# Autodesk Inventor assembly: Motors with Screws
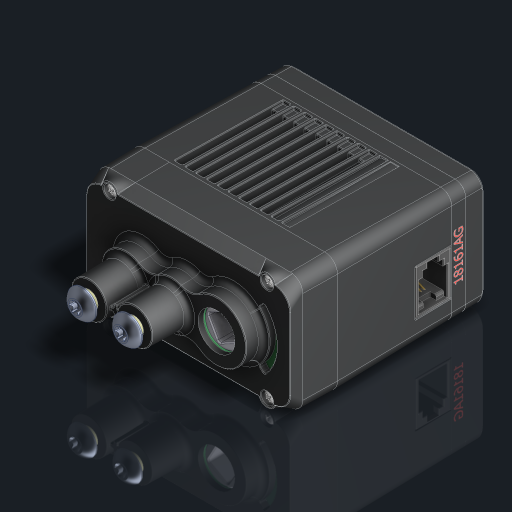
[picture p0: Inventor's stored thumbnail of the model, 512x512]
Saved by Autodesk Inventor 2023.2 (Build 272271030, 271C)
## iProperties
Created: 2022-08-18
Part Number: Motors with Screws
Document SubType Name: Assembly
Designer: ylu12
Author: ylu12
## Documents named in this file (5)
- C:\Users\black\OneDrive\Pictures\Documents\GitHub\New folder\2024-599Z\Cad\Library\VEX-CAD-Inventor-1.4.0\Electronics\Motors with Screws\AluM-StarS.iam
- C:\Users\black\OneDrive\Pictures\Documents\GitHub\New folder\2024-599Z\Cad\Library\VEX-CAD-Inventor-1.4.0\Electronics\V5 Motor.ipt
- C:\Users\black\OneDrive\Pictures\Documents\GitHub\New folder\2024-599Z\Cad\Library\VEX-CAD-Inventor-1.4.0\Structure\Hardware\Screw Steel - Star\SScrew Star Smooth .500.ipt
- C:\Users\black\OneDrive\Pictures\Documents\GitHub\New folder\2024-599Z\Cad\Library\VEX-CAD-Inventor-1.4.0\Structure\Hardware\Screw Steel - Star.ipt
- C:\Users\black\OneDrive\Pictures\Documents\GitHub\New folder\2024-599Z\Cad\Library\VEX-CAD-Inventor-1.4.0\Electronics\Motors with Screws.iam
## Components (3 placed, 2 different names)
1. V5 Motor:1
2. SScrew Star Smooth .500:1
3. SScrew Star Smooth .500:2
## Named parameters: Thickness = 1.5875 mm
